# Autodesk Inventor assembly: Final Project Assem
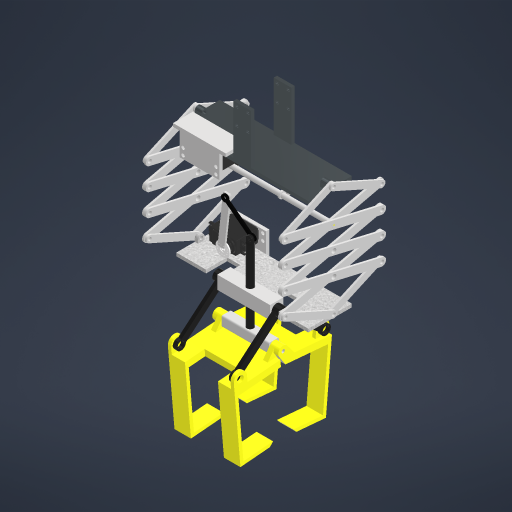
[picture p0: Inventor's stored thumbnail of the model, 512x512]
Saved by Autodesk Inventor 2023.6 (Build 276521000, 521)
## iProperties
Created: 2026-03-02
Part Number: Final Project Assem
Document SubType Name: Assembly
Designer: user
Author: user
## Documents named in this file (17)
- D:\FP (Sebelum Revisi)\Final Project Assem.iam
- D:\FP (Sebelum Revisi)\FP V2 Claw.ipt
- D:\FP (Sebelum Revisi)\FP V2 Claw_Side.ipt
- D:\FP (Sebelum Revisi)\FP V2 Claw Connector.ipt
- D:\FP (Sebelum Revisi)\FP V2 Shaft.ipt
- D:\FP (Sebelum Revisi)\FP V2 Arm Connector.ipt
- D:\FP (Sebelum Revisi)\FP V2 Lengan Serok.ipt
- D:\FP (Sebelum Revisi)\FP V2 Mounting Claw.ipt
- D:\FP (Sebelum Revisi)\FP V2 Spring beam Short.ipt
- D:\FP (Sebelum Revisi)\FP V2 Spring Beam.ipt
- D:\FP (Sebelum Revisi)\FP V2 Mounting Plate.ipt
- D:\FP (Sebelum Revisi)\FP V2 Z Axis connector.ipt
- D:\FP (Sebelum Revisi)\FP V2 Spring Beam connector.ipt
- D:\FP (Sebelum Revisi)\fp v2 servo Mounting.ipt
- D:\FP (Sebelum Revisi)\MG_996R.iam
- D:\FP (Sebelum Revisi)\FP V2 Batang Penggerak.ipt
- D:\FP (Sebelum Revisi)\MG_996R v1.iam
## Components (38 placed, 16 different names)
1. FP V2 Claw Connector:1 — Mate:5, Mate:6, Mate:101, Mate:102
2. FP V2 Shaft:1 — Mate:5, Mate:6, Mate:7, Mate:86, Mate:88
3. FP V2 Arm Connector:1 — Mate:7, Mate:20, Mate:21, Flush:5, Mate:105, Mate:110, Mate:112, Mate:115
4. FP V2 Mounting Claw:1 — Mate:20, Mate:21, Mate:77, Mate:78, Mate:79, Mate:80, Mate:81, Flush:2, Flush:5, Flush:6
5. FP V2 Spring beam Short:2 — Mate:41, Mate:42, Mate:44, Mate:68
6. FP V2 Spring beam Short:3 — Mate:40, Mate:43, Mate:44, Mate:67
7. FP V2 Spring Beam:1 — Mate:23, Mate:24, Mate:25, Mate:28, Mate:32, Mate:33
8. FP V2 Spring Beam:2 — Mate:30, Mate:31, Mate:34, Mate:35, Mate:37
9. FP V2 Spring Beam:3 — Mate:23, Mate:24, Mate:26, Mate:27, Mate:30, Mate:31, Mate:75
10. FP V2 Spring Beam:4 — Mate:32, Mate:33, Mate:34, Mate:36, Mate:38, Mate:74
11. FP V2 Spring Beam:5 — Mate:36, Mate:38, Mate:39, Mate:40, Mate:43
12. FP V2 Spring Beam:6 — Mate:35, Mate:37, Mate:39, Mate:41, Mate:42, Mate:72, Flush:4
13. FP V2 Spring beam Short:4 — Mate:25, Mate:28, Mate:29, Mate:76, Mate:77
14. FP V2 Spring beam Short:5 — Mate:26, Mate:27, Mate:29
15. FP V2 Spring beam Short:6
16. FP V2 Spring beam Short:7 — Mate:69, Mate:70
17. FP V2 Spring Beam:7
18. FP V2 Spring Beam:8
19. FP V2 Spring Beam:9 — Mate:75
20. FP V2 Spring Beam:10 — Mate:74
21. FP V2 Spring Beam:11
22. FP V2 Spring Beam:12 — Mate:73
23. FP V2 Spring beam Short:8 — Mate:76, Mate:78, Mate:79
24. FP V2 Spring beam Short:9
25. FP V2 Mounting Plate:1 — Mate:67, Mate:68, Mate:69, Mate:70, Mate:90, Mate:91, Flush:3, Flush:6
26. FP V2 Z Axis connector:1 — Mate:92, Mate:98
27. FP V2 Spring Beam connector:1 — Mate:72, Mate:73, Mate:92, Flush:4
28. fp v2 servo Mounting:1 — Mate:80, Mate:81, Flush:2, Mate:82, Mate:83, Mate:84, Mate:85
29. fp v2 servo Mounting:2 — Mate:90, Mate:91, Flush:3, Mate:93, Mate:94, Mate:95, Mate:96, Mate:97
30. MG_996R:1 [sub-assembly] — Mate:82, Mate:83, Mate:84, Mate:85, Mate:87
31. FP V2 Batang Penggerak:1 — Mate:86, Mate:87, Mate:88
32. MG_996R v1:1 [sub-assembly] — Mate:93, Mate:94, Mate:95, Mate:96, Mate:97, Mate:98
33. FP V2 Claw:1 — Mate:99, Mate:100, Mate:101, Mate:108, Mate:109, Mate:116, Mate:117
34. FP V2 Claw_Side:1 — Mate:99, Mate:100, Mate:102, Mate:106, Mate:107, Mate:113, Mate:114
35. FP V2 Lengan Serok:1 — Mate:105, Mate:106, Mate:107
36. FP V2 Lengan Serok:2 — Mate:111, Mate:112, Mate:113, Mate:114
37. FP V2 Lengan Serok:4 — Mate:111, Mate:115, Mate:116, Mate:117
38. FP V2 Lengan Serok:5 — Mate:108, Mate:109, Mate:110
## Relationships (101: Mate 96, Flush 5)
- Mate:5: FP V2 Claw Connector:1 ↔ FP V2 Shaft:1
- Mate:6: FP V2 Claw Connector:1 ↔ FP V2 Shaft:1
- Mate:7: FP V2 Shaft:1 ↔ FP V2 Arm Connector:1
- Mate:20: FP V2 Arm Connector:1 ↔ FP V2 Mounting Claw:1
- Mate:21 (5 mm): FP V2 Arm Connector:1 ↔ FP V2 Mounting Claw:1
- Mate:23: FP V2 Spring Beam:1 ↔ FP V2 Spring Beam:3
- Mate:24: FP V2 Spring Beam:1 ↔ FP V2 Spring Beam:3
- Mate:25: FP V2 Spring Beam:1 ↔ FP V2 Spring beam Short:4
- Mate:26: FP V2 Spring Beam:3 ↔ FP V2 Spring beam Short:5
- Mate:27: FP V2 Spring Beam:3 ↔ FP V2 Spring beam Short:5
- Mate:28: FP V2 Spring Beam:1 ↔ FP V2 Spring beam Short:4
- Mate:29: FP V2 Spring beam Short:4 ↔ FP V2 Spring beam Short:5
- Mate:30: FP V2 Spring Beam:2 ↔ FP V2 Spring Beam:3
- Mate:31: FP V2 Spring Beam:2 ↔ FP V2 Spring Beam:3
- Mate:32: FP V2 Spring Beam:1 ↔ FP V2 Spring Beam:4
- Mate:33: FP V2 Spring Beam:1 ↔ FP V2 Spring Beam:4
- Mate:34: FP V2 Spring Beam:2 ↔ FP V2 Spring Beam:4
- Mate:35: FP V2 Spring Beam:2 ↔ FP V2 Spring Beam:6
- Mate:36: FP V2 Spring Beam:4 ↔ FP V2 Spring Beam:5
- Mate:37: FP V2 Spring Beam:2 ↔ FP V2 Spring Beam:6
- Mate:38: FP V2 Spring Beam:4 ↔ FP V2 Spring Beam:5
- Mate:39: FP V2 Spring Beam:5 ↔ FP V2 Spring Beam:6
- Mate:40: FP V2 Spring beam Short:3 ↔ FP V2 Spring Beam:5
- Mate:41: FP V2 Spring beam Short:2 ↔ FP V2 Spring Beam:6
- Mate:42: FP V2 Spring beam Short:2 ↔ FP V2 Spring Beam:6
- Mate:43: FP V2 Spring beam Short:3 ↔ FP V2 Spring Beam:5
- Mate:44: FP V2 Spring beam Short:2 ↔ FP V2 Spring beam Short:3
- [Mate]: FP V2 Spring Beam:7 ↔ FP V2 Spring Beam:9
- [Mate]: FP V2 Spring Beam:7 ↔ FP V2 Spring Beam:9
- [Mate]: FP V2 Spring Beam:7 ↔ FP V2 Spring beam Short:8
- [Mate]: FP V2 Spring Beam:9 ↔ FP V2 Spring beam Short:9
- [Mate]: FP V2 Spring Beam:9 ↔ FP V2 Spring beam Short:9
- [Mate]: FP V2 Spring Beam:7 ↔ FP V2 Spring beam Short:8
- [Mate]: FP V2 Spring beam Short:8 ↔ FP V2 Spring beam Short:9
- [Mate]: FP V2 Spring Beam:8 ↔ FP V2 Spring Beam:9
- [Mate]: FP V2 Spring Beam:8 ↔ FP V2 Spring Beam:9
- [Mate]: FP V2 Spring Beam:7 ↔ FP V2 Spring Beam:10
- [Mate]: FP V2 Spring Beam:7 ↔ FP V2 Spring Beam:10
- [Mate]: FP V2 Spring Beam:8 ↔ FP V2 Spring Beam:10
- [Mate]: FP V2 Spring Beam:8 ↔ FP V2 Spring Beam:12
- [Mate]: FP V2 Spring Beam:10 ↔ FP V2 Spring Beam:11
- [Mate]: FP V2 Spring Beam:8 ↔ FP V2 Spring Beam:12
- [Mate]: FP V2 Spring Beam:10 ↔ FP V2 Spring Beam:11
- [Mate]: FP V2 Spring Beam:11 ↔ FP V2 Spring Beam:12
- [Mate]: FP V2 Spring beam Short:7 ↔ FP V2 Spring Beam:11
- [Mate]: FP V2 Spring beam Short:6 ↔ FP V2 Spring Beam:12
- [Mate]: FP V2 Spring beam Short:6 ↔ FP V2 Spring Beam:12
- [Mate]: FP V2 Spring beam Short:7 ↔ FP V2 Spring Beam:11
- [Mate]: FP V2 Spring beam Short:6 ↔ FP V2 Spring beam Short:7
- Mate:67: FP V2 Spring beam Short:3 ↔ FP V2 Mounting Plate:1
- Mate:68: FP V2 Spring beam Short:2 ↔ FP V2 Mounting Plate:1
- Mate:69: FP V2 Spring beam Short:7 ↔ FP V2 Mounting Plate:1
- Mate:70: FP V2 Spring beam Short:7 ↔ FP V2 Mounting Plate:1
- Mate:72: FP V2 Spring Beam:6 ↔ FP V2 Spring Beam connector:1
- Mate:73: FP V2 Spring Beam:12 ↔ FP V2 Spring Beam connector:1
- Mate:74: FP V2 Spring Beam:4 ↔ FP V2 Spring Beam:10
- Mate:75: FP V2 Spring Beam:3 ↔ FP V2 Spring Beam:9
- Mate:76: FP V2 Spring beam Short:4 ↔ FP V2 Spring beam Short:8
- Mate:77: FP V2 Mounting Claw:1 ↔ FP V2 Spring beam Short:4
- Mate:78: FP V2 Mounting Claw:1 ↔ FP V2 Spring beam Short:8
- Mate:79: FP V2 Mounting Claw:1 ↔ FP V2 Spring beam Short:8
- Mate:80: FP V2 Mounting Claw:1 ↔ fp v2 servo Mounting:1
- Mate:81: FP V2 Mounting Claw:1 ↔ fp v2 servo Mounting:1
- Flush:2: FP V2 Mounting Claw:1 ↔ fp v2 servo Mounting:1
- Mate:82: fp v2 servo Mounting:1 ↔ MG_996R:1
- Mate:83: fp v2 servo Mounting:1 ↔ MG_996R:1
- Mate:84: fp v2 servo Mounting:1 ↔ MG_996R:1
- Mate:85: fp v2 servo Mounting:1 ↔ MG_996R:1
- Mate:86: FP V2 Shaft:1 ↔ FP V2 Batang Penggerak:1
- Mate:87: MG_996R:1 ↔ FP V2 Batang Penggerak:1
- Mate:88: FP V2 Shaft:1 ↔ FP V2 Batang Penggerak:1
- Mate:90: FP V2 Mounting Plate:1 ↔ fp v2 servo Mounting:2
- Mate:91: FP V2 Mounting Plate:1 ↔ fp v2 servo Mounting:2
- Flush:3: FP V2 Mounting Plate:1 ↔ fp v2 servo Mounting:2
- Mate:92: FP V2 Z Axis connector:1 ↔ FP V2 Spring Beam connector:1
- Mate:93: fp v2 servo Mounting:2 ↔ MG_996R v1:1
- Mate:94: fp v2 servo Mounting:2 ↔ MG_996R v1:1
- Mate:95: fp v2 servo Mounting:2 ↔ MG_996R v1:1
- Mate:96: fp v2 servo Mounting:2 ↔ MG_996R v1:1
- Mate:97: fp v2 servo Mounting:2 ↔ MG_996R v1:1
- Flush:4: FP V2 Spring Beam:6 ↔ FP V2 Spring Beam connector:1
- Mate:98: FP V2 Z Axis connector:1 ↔ MG_996R v1:1
- Flush:5: FP V2 Arm Connector:1 ↔ FP V2 Mounting Claw:1
- Flush:6: FP V2 Mounting Claw:1 ↔ FP V2 Mounting Plate:1
- Mate:99: FP V2 Claw:1 ↔ FP V2 Claw_Side:1
- Mate:100: FP V2 Claw:1 ↔ FP V2 Claw_Side:1
- Mate:101: FP V2 Claw Connector:1 ↔ FP V2 Claw:1
- Mate:102: FP V2 Claw Connector:1 ↔ FP V2 Claw_Side:1
- Mate:105: FP V2 Arm Connector:1 ↔ FP V2 Lengan Serok:1
- Mate:106: FP V2 Claw_Side:1 ↔ FP V2 Lengan Serok:1
- Mate:107: FP V2 Claw_Side:1 ↔ FP V2 Lengan Serok:1
- Mate:108: FP V2 Claw:1 ↔ FP V2 Lengan Serok:5
- Mate:109: FP V2 Claw:1 ↔ FP V2 Lengan Serok:5
- Mate:110: FP V2 Arm Connector:1 ↔ FP V2 Lengan Serok:5
- Mate:111: FP V2 Lengan Serok:2 ↔ FP V2 Lengan Serok:4
- Mate:112: FP V2 Arm Connector:1 ↔ FP V2 Lengan Serok:2
- Mate:113: FP V2 Claw_Side:1 ↔ FP V2 Lengan Serok:2
- Mate:114: FP V2 Claw_Side:1 ↔ FP V2 Lengan Serok:2
- Mate:115: FP V2 Arm Connector:1 ↔ FP V2 Lengan Serok:4
- Mate:116: FP V2 Claw:1 ↔ FP V2 Lengan Serok:4
- Mate:117: FP V2 Claw:1 ↔ FP V2 Lengan Serok:4
## Named parameters: d48_d26 = 0 mm, d49_d27 = 0 mm, d50_d28 = 0 mm, d51_d29 = 0 mm, d52_d30 = 0 mm, d53_d31 = 0 mm, d54_d32 = 0 mm, d55_d33 = 0 mm, d56_d34 = 0 mm, d57_d35 = 0 mm, d58_d36 = 0 mm, d59_d37 = 0 mm, d60_d38 = 0 mm, d61_d39 = 0 mm, d62_d40 = 0 mm, d63_d41 = 0 mm, d64_d42 = 0 mm, d65_d43 = 0 mm, d66_d44 = 0 mm, d67_d45 = 0 mm, d68_d46 = 0 mm, d69_d47 = 0 mm
